# Autodesk Inventor assembly: Drifter_Assembly
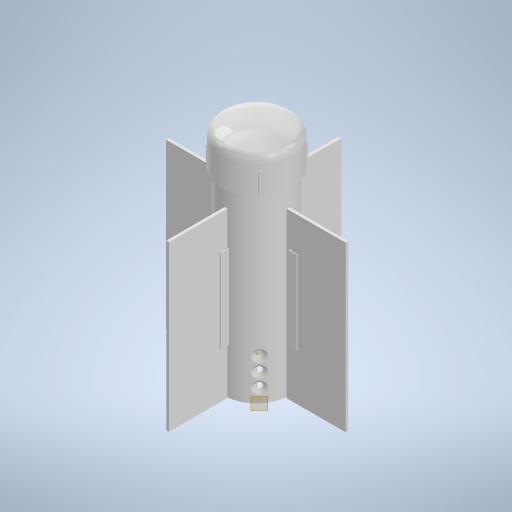
[picture p0: Inventor's stored thumbnail of the model, 512x512]
Saved by Autodesk Inventor 2024 (Build 280153000, 153)
## iProperties
Created: 2024-05-17
Part Number: Drifter_Assembly
Document SubType Name: Assembly
Designer: sml6042
Author: sml6042
## Documents named in this file (5)
- C:\Users\sml6042\Documents\Drifter_Assembly.iam
- C:\Users\sml6042\Documents\Drifter_Body.ipt
- C:\Users\sml6042\Downloads\4880K811_Standard-Wall PVC Pipe Fitting for Water\4880K811_Standard-Wall PVC Pipe Fitting for Water.ipt
- C:\Users\sml6042\Downloads\85065K33_Chemical-Resistant PVC U-Channel\85065K33_Chemical-Resistant PVC U-Channel.ipt
- C:\Users\sml6042\Documents\Drag_Vane.ipt
## Components (10 placed, 4 different names)
1. Drifter_Body:1 — Rigid:1, Mate:1, Flush:1, Tangent:1, Mate:2, Flush:2, Tangent:2, Flush:3, Flush:4
2. 4880K811_Standard-Wall PVC Pipe Fitting for Water:1 — Rigid:1
3. 85065K33_Chemical-Resistant PVC U-Channel:1 — Flush:2, Tangent:2
4. 85065K33_Chemical-Resistant PVC U-Channel:2
5. 85065K33_Chemical-Resistant PVC U-Channel:3 — Rigid:2, Rigid:3
6. 85065K33_Chemical-Resistant PVC U-Channel:4 — Mate:1, Flush:1, Tangent:1
7. Drag_Vane:1
8. Drag_Vane:2 — Rigid:2, Rigid:3, Flush:4
9. Drag_Vane:3
10. Drag_Vane:4 — Flush:3
## Relationships (11: Flush 4, WeldJoint 3, Mate 2, Tangent 2)
- Rigid:1 [WeldJoint]: Drifter_Body:1 ↔ 4880K811_Standard-Wall PVC Pipe Fitting for Water:1
- Mate:1 (100 mm): Drifter_Body:1 ↔ 85065K33_Chemical-Resistant PVC U-Channel:4
- Flush:1 (85 mm): Drifter_Body:1 ↔ 85065K33_Chemical-Resistant PVC U-Channel:4
- Tangent:1: Drifter_Body:1 ↔ 85065K33_Chemical-Resistant PVC U-Channel:4
- Mate:2: Drifter_Body:1
- Flush:2 (85 mm): Drifter_Body:1 ↔ 85065K33_Chemical-Resistant PVC U-Channel:1
- Tangent:2: Drifter_Body:1 ↔ 85065K33_Chemical-Resistant PVC U-Channel:1
- Rigid:2 [WeldJoint]: 85065K33_Chemical-Resistant PVC U-Channel:3 ↔ Drag_Vane:2
- Flush:3: Drifter_Body:1 ↔ Drag_Vane:4
- Rigid:3 [WeldJoint]: 85065K33_Chemical-Resistant PVC U-Channel:3 ↔ Drag_Vane:2
- Flush:4: Drifter_Body:1 ↔ Drag_Vane:2
